# Autodesk Inventor assembly: Storage Tank
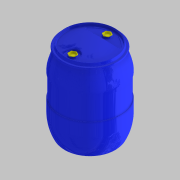
[picture p0: Inventor's stored thumbnail of the model, 180x180]
Saved by Autodesk Inventor 2020 (Build 240168000, 168)
## iProperties
Created: 2020-06-20
Part Number: Storage Tank
Document SubType Name: Assembly
Designer: Abbas
Sending System: Autodesk Inventor 2020
Preprocessor: ST-DEVELOPER v18
Title: C:\Users\Administrator\Documents\55 gallon barrel cap assy.stp
Author: Administrator
## Documents named in this file (4)
- C:\Users\LENOVO\Desktop\Graduation Project\Fish Farming Unit\Water Loop Components\55-gallon-barrel-1.snapshot.3\Storage Tank.iam
- C:\Users\LENOVO\Desktop\Graduation Project\Fish Farming Unit\Water Loop Components\55-gallon-barrel-1.snapshot.3\55 gallon barrel cap.ipt
- C:\Users\LENOVO\Desktop\Graduation Project\Fish Farming Unit\Water Loop Components\55-gallon-barrel-1.snapshot.3\PLUG_2in_-_Yellow.ipt
- C:\Users\LENOVO\Desktop\Graduation Project\Fish Farming Unit\Water Loop Components\55-gallon-barrel-1.snapshot.3\User Library-55 Gallon Water Barrel_.ipt
## Components (4 placed, 3 different names)
1. 55 gallon barrel cap:1 — Mate:1
2. PLUG_2in_-_Yellow:1
3. PLUG_2in_-_Yellow:2
4. User Library-55 Gallon Water Barrel_:1 — Mate:1
## Relationships (1: Mate 1)
- Mate:1: 55 gallon barrel cap:1 ↔ User Library-55 Gallon Water Barrel_:1
